# Autodesk Inventor assembly: rev2 base
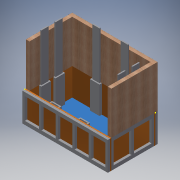
[picture p0: Inventor's stored thumbnail of the model, 180x180]
Saved by Autodesk Inventor 2017 (Build 210142000, 142)
## iProperties
Created: 2019-05-04
Part Number: rev2 base
Document SubType Name: Assembly
Designer: Roman
Author: Roman
## Documents named in this file (6)
- C:\Users\Roman\Documents\CAD\enclosure rev1\rev2 base\rev2 base.iam
- C:\Users\Roman\Documents\CAD\enclosure rev1\rev2 base\rev1 large wall\rev1 base large wall.iam
- C:\Users\Roman\Documents\CAD\enclosure rev1\rev2 base\rev1 small wall\rev1 base short wall.iam
- C:\Users\Roman\Documents\CAD\enclosure rev1\rev2 base\rev1 base floor.ipt
- C:\Users\Roman\Documents\CAD\enclosure rev1\rev2 large wall\rev2 top large wall.iam
- C:\Users\Roman\Documents\CAD\enclosure rev1\rev2 short wall\rev2 top short wall.iam
## Components (8 placed, 5 different names)
1. rev1 base large wall:1 [sub-assembly] — Mate:1, Flush:1, Flush:2, Flush:5, Mate:3, Flush:10
2. rev1 base short wall:1 [sub-assembly] — Mate:1, Flush:1, Flush:2, Mate:14, Mate:15
3. rev1 base short wall:2 [sub-assembly] — Flush:5, Mate:3, Flush:8, Mate:5, Flush:9, Flush:10, Mate:6, Flush:11, Mate:12, Mate:13
4. rev1 base large wall:2 [sub-assembly] — Flush:8, Mate:5, Flush:9, Mate:7, Mate:9, Flush:12
5. rev1 base floor:1 — Mate:6, Flush:11, Mate:7, Mate:8, Mate:10, Mate:11
6. rev2 top large wall:1 [sub-assembly] — Mate:8, Mate:9, Flush:12
7. rev2 top short wall:1 [sub-assembly] — Mate:10, Mate:12, Mate:13
8. rev2 top short wall:2 [sub-assembly] — Mate:11, Mate:14, Mate:15
## Relationships (21: Mate 13, Flush 8)
- Mate:1: rev1 base large wall:1 ↔ rev1 base short wall:1
- Flush:1: rev1 base large wall:1 ↔ rev1 base short wall:1
- Flush:2: rev1 base large wall:1 ↔ rev1 base short wall:1
- Flush:5: rev1 base large wall:1 ↔ rev1 base short wall:2
- Mate:3: rev1 base large wall:1 ↔ rev1 base short wall:2
- Flush:8: rev1 base short wall:2 ↔ rev1 base large wall:2
- Mate:5: rev1 base short wall:2 ↔ rev1 base large wall:2
- Flush:9: rev1 base short wall:2 ↔ rev1 base large wall:2
- Flush:10: rev1 base large wall:1 ↔ rev1 base short wall:2
- Mate:6: rev1 base short wall:2 ↔ rev1 base floor:1
- Flush:11: rev1 base short wall:2 ↔ rev1 base floor:1
- Mate:7: rev1 base large wall:2 ↔ rev1 base floor:1
- Mate:8: rev1 base floor:1 ↔ rev2 top large wall:1
- Mate:9: rev1 base large wall:2 ↔ rev2 top large wall:1
- Flush:12: rev1 base large wall:2 ↔ rev2 top large wall:1
- Mate:10: rev1 base floor:1 ↔ rev2 top short wall:1
- Mate:11: rev1 base floor:1 ↔ rev2 top short wall:2
- Mate:12: rev1 base short wall:2 ↔ rev2 top short wall:1
- Mate:13: rev1 base short wall:2 ↔ rev2 top short wall:1
- Mate:14: rev1 base short wall:1 ↔ rev2 top short wall:2
- Mate:15: rev1 base short wall:1 ↔ rev2 top short wall:2
